# Autodesk Inventor assembly: Slide rod assembly
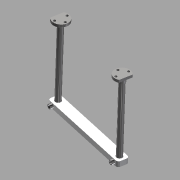
[picture p0: Inventor's stored thumbnail of the model, 180x180]
Saved by Autodesk Inventor 2017 (Build 210142000, 142)
## iProperties
Created: 2016-12-06
Part Number: Slide rod assembly
Document SubType Name: Assembly
Designer: qupec
Author: qupec
## Documents named in this file (4)
- C:\Users\qupec\Desktop\UMD Near Space\STAR\CAD\Mechanical\Slide rod assembly.iam
- C:\Users\qupec\Desktop\UMD Near Space\STAR\CAD\Mechanical\Slide rod connector.ipt
- C:\Users\qupec\Desktop\UMD Near Space\STAR\CAD\Mechanical\slide rod.ipt
- C:\Users\qupec\Desktop\UMD Near Space\STAR\CAD\Mechanical\Slide rod set screw.ipt
## Components (5 placed, 3 different names)
1. Slide rod connector:1 — Mate:1, Mate:11, Mate:12, Mate:15, Mate:16, Flush:1, Flush:2, Mate:18
2. slide rod:1 — Mate:11, Mate:14, Flush:2, Mate:17, Mate:18
3. slide rod:2 — Mate:1, Mate:12, Mate:13, Flush:1
4. Slide rod set screw:1 — Mate:13, Mate:16
5. Slide rod set screw:2 — Mate:14, Mate:15, Mate:17
## Relationships (11: Mate 9, Flush 2)
- Mate:1: Slide rod connector:1 ↔ slide rod:2
- Mate:11: Slide rod connector:1 ↔ slide rod:1
- Mate:12: Slide rod connector:1 ↔ slide rod:2
- Mate:13: slide rod:2 ↔ Slide rod set screw:1
- Mate:14: slide rod:1 ↔ Slide rod set screw:2
- Mate:15: Slide rod connector:1 ↔ Slide rod set screw:2
- Mate:16: Slide rod connector:1 ↔ Slide rod set screw:1
- Flush:1: Slide rod connector:1 ↔ slide rod:2
- Flush:2: Slide rod connector:1 ↔ slide rod:1
- Mate:17: slide rod:1 ↔ Slide rod set screw:2
- Mate:18: Slide rod connector:1 ↔ slide rod:1
